# Autodesk Inventor assembly: ASY MSC 100 CONE
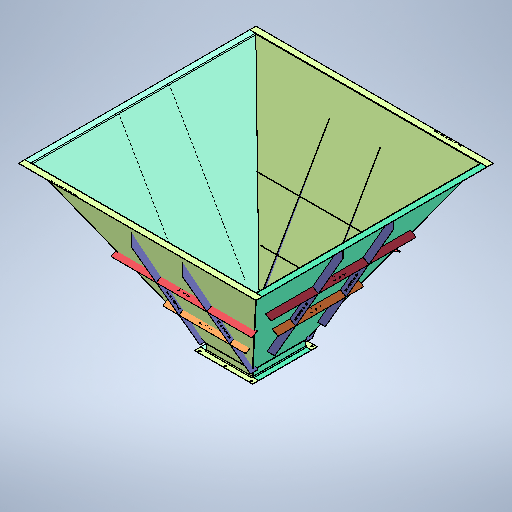
[picture p0: Inventor's stored thumbnail of the model, 512x512]
Saved by Autodesk Inventor 2025.1 (Build 291241020, 241B)
## iProperties
Created: 2024-05-19
Part Number: ASY MSC 100 CONE
Document SubType Name: Assembly
Designer: admin
Mass: 170206 g
Surface Area: 120081 cm^2
Volume: 21304.1 cm^3
Density: 7.98935 g/cm^3
Stock Number: ASY МОО 100 конус
Author: admin
## Documents named in this file (12)
- C:\Users\user\YandexDisk-badmisterfox\домашниий пк\Inventor\NDM-VOS_powder_hopper\Workspaces\Workspace\Cone\ASY MSC 100 cone.iam
- C:\Users\user\YandexDisk-badmisterfox\домашниий пк\Inventor\NDM-VOS_powder_hopper\Workspaces\Workspace\Cone\MSC 114 cone IN right board.ipt
- C:\Users\user\YandexDisk-badmisterfox\домашниий пк\Inventor\NDM-VOS_powder_hopper\Workspaces\Workspace\Cone\MSC 113 cone IN left board.ipt
- C:\Users\user\YandexDisk-badmisterfox\домашниий пк\Inventor\NDM-VOS_powder_hopper\Workspaces\Workspace\Cone\MSC 112 cone IN back.ipt
- C:\Users\user\YandexDisk-badmisterfox\домашниий пк\Inventor\NDM-VOS_powder_hopper\Workspaces\Workspace\Cone\MSC DIM 001 cone sketch.ipt
- C:\Users\user\YandexDisk-badmisterfox\домашниий пк\Inventor\NDM-VOS_powder_hopper\Workspaces\Workspace\Cone\MSC 115 cone IN bow.ipt
- C:\Users\user\YandexDisk-badmisterfox\домашниий пк\Inventor\NDM-VOS_powder_hopper\Workspaces\Workspace\Cone\MSC 110 stringer cone.ipt
- C:\Users\user\YandexDisk-badmisterfox\домашниий пк\Inventor\NDM-VOS_powder_hopper\Workspaces\Workspace\Cone\MSC 106 rib cone.ipt
- C:\Users\user\YandexDisk-badmisterfox\домашниий пк\Inventor\NDM-VOS_powder_hopper\Workspaces\Workspace\Cone\MSC 107 rib cone.ipt
- C:\Users\user\YandexDisk-badmisterfox\домашниий пк\Inventor\NDM-VOS_powder_hopper\Workspaces\Workspace\Cone\MSC 108 rib cone.ipt
- C:\Users\user\YandexDisk-badmisterfox\домашниий пк\Inventor\NDM-VOS_powder_hopper\Workspaces\Workspace\Cone\MSC 109 rib cone.ipt
- C:\Users\user\YandexDisk-badmisterfox\домашниий пк\Inventor\NDM-VOS_powder_hopper\NDM-VOS dummy2.ipt
## Components (23 placed, 12 different names)
1. NDM-VOS dummy2:1 — Mate:73, Mate:74, Flush:19
2. MSC DIM 001 CONE SKETCH:1 — Flush:8, Flush:9, Mate:1
3. MSC 112 CONE IN BACK:1 — Flush:6, Flush:10, Mate:2, Mate:49, Mate:70, Mate:72
4. MSC 114 CONE IN RIGHT BOARD:1 — Flush:13, Flush:15, Mate:63, Mate:66, Mate:67, Mate:68, Mate:69, Flush:18
5. MSC 113 CONE IN LEFT BOARD:1 — Mate:4, Flush:14, Mate:5
6. MSC 115 CONE IN BOW:1 — Mate:6, Flush:16, Flush:17
7. MSC 115 cone IN bow:2 — Mate:75, Flush:20, Flush:21
8. MSC 110 STRINGER CONE:1 — Rigid:7
9. MSC 107 RIB CONE:1 — Rigid:9
10. MSC 110 STRINGER CONE:2 — Mate:49, Rigid:8, Rigid:9, Mate:72
11. MSC 110 STRINGER CONE:3 — Rigid:5
12. MSC 108 RIB CONE:1 — Mate:66, Rigid:4, Rigid:5, Mate:67, Mate:68
13. MSC 110 STRINGER CONE:4 — Rigid:4, Rigid:6, Mate:69
14. MSC 109 RIB CONE:1 — Mate:63, Rigid:6
15. MSC 106 RIB CONE:1 — Rigid:7, Rigid:8, Mate:70, Mate:71
16. MSC 110 STRINGER CONE:5
17. MSC 107 RIB CONE:2
18. MSC 110 STRINGER CONE:6
19. MSC 110 STRINGER CONE:7
20. MSC 108 RIB CONE:2
21. MSC 110 STRINGER CONE:8
22. MSC 109 RIB CONE:2
23. MSC 106 RIB CONE:2
## Component patterns: (2 elements, first: MSC 110 STRINGER CONE:1 + MSC 107 RIB CONE:1 + MSC 110 STRINGER CONE:2 + MSC 110 STRINGER CONE:3 + MSC 108 RIB CONE:1 + MSC 110 STRINGER CONE:4 + MSC 109 RIB CONE:1 + MSC 106 RIB CONE:1)
## Relationships (36: Mate 17, Flush 13, WeldJoint 6)
- Flush:6: MSC 112 CONE IN BACK:1
- Flush:8: MSC DIM 001 CONE SKETCH:1
- Flush:9: MSC DIM 001 CONE SKETCH:1
- Mate:1: MSC DIM 001 CONE SKETCH:1
- Flush:10: MSC 112 CONE IN BACK:1
- Mate:2: MSC 112 CONE IN BACK:1
- Flush:13: MSC 114 CONE IN RIGHT BOARD:1
- Mate:4: MSC 113 CONE IN LEFT BOARD:1
- Flush:14: MSC 113 CONE IN LEFT BOARD:1
- Mate:5: MSC 113 CONE IN LEFT BOARD:1
- Flush:15: MSC 114 CONE IN RIGHT BOARD:1
- Mate:6: MSC 115 CONE IN BOW:1
- Flush:16: MSC 115 CONE IN BOW:1
- Flush:17: MSC 115 CONE IN BOW:1
- Mate:49: MSC 112 CONE IN BACK:1 ↔ MSC 110 STRINGER CONE:2
- Mate:63: MSC 114 CONE IN RIGHT BOARD:1 ↔ MSC 109 RIB CONE:1
- Mate:66: MSC 114 CONE IN RIGHT BOARD:1 ↔ MSC 108 RIB CONE:1
- Rigid:4 [WeldJoint] (2 mm): MSC 108 RIB CONE:1 ↔ MSC 110 STRINGER CONE:4
- Rigid:5 [WeldJoint] (2 mm): MSC 110 STRINGER CONE:3 ↔ MSC 108 RIB CONE:1
- Rigid:6 [WeldJoint] (2 mm): MSC 110 STRINGER CONE:4 ↔ MSC 109 RIB CONE:1
- Mate:67: MSC 114 CONE IN RIGHT BOARD:1 ↔ MSC 108 RIB CONE:1
- Mate:68: MSC 114 CONE IN RIGHT BOARD:1 ↔ MSC 108 RIB CONE:1
- Mate:69 (5 mm): MSC 114 CONE IN RIGHT BOARD:1 ↔ MSC 110 STRINGER CONE:4
- Rigid:7 [WeldJoint] (3 mm): MSC 110 STRINGER CONE:1 ↔ MSC 106 RIB CONE:1
- Rigid:8 [WeldJoint] (2 mm): MSC 110 STRINGER CONE:2 ↔ MSC 106 RIB CONE:1
- Rigid:9 [WeldJoint] (2 mm): MSC 107 RIB CONE:1 ↔ MSC 110 STRINGER CONE:2
- Mate:70: MSC 112 CONE IN BACK:1 ↔ MSC 106 RIB CONE:1
- Flush:18: MSC 114 CONE IN RIGHT BOARD:1
- Mate:71: MSC 106 RIB CONE:1
- Mate:72 (5 mm): MSC 112 CONE IN BACK:1 ↔ MSC 110 STRINGER CONE:2
- Mate:73: NDM-VOS dummy2:1
- Mate:74: NDM-VOS dummy2:1
- Flush:19: NDM-VOS dummy2:1
- Mate:75: MSC 115 cone IN bow:2
- Flush:20: MSC 115 cone IN bow:2
- Flush:21: MSC 115 cone IN bow:2
## Named parameters: Конус_Базовая_Высота = 1170 mm, Конус_отступ_от_пола = 0 mm
